# Autodesk Inventor assembly: MaleHeaderPin_1x2
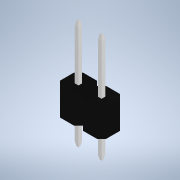
[picture p0: Inventor's stored thumbnail of the model, 180x180]
Saved by Autodesk Inventor 2021 (Build 250183000, 183)
## iProperties
Created: 2020-01-06
Part Number: MaleHeaderPin_1x2
Document SubType Name: Assembly
Designer: ermoz
Author: ermoz
## Documents named in this file (2)
- D:\Moje Wyczyny\My_Poor_Projects\Sneak100_MiniSumo\minisumo-sneak100\mechanics\PreMadeParts\MaleHeaderPin_1x2.iam
- D:\Moje Wyczyny\My_Poor_Projects\Sneak100_MiniSumo\minisumo-sneak100\mechanics\PreMadeParts\MaleHeaderPin.ipt
## Components (2 placed, 1 different names)
1. MaleHeaderPin:1 — Flush:1, Flush:8, Mate:1
2. MaleHeaderPin:2 — Flush:1, Flush:8, Mate:1
## Relationships (3: Flush 2, Mate 1)
- Flush:1: MaleHeaderPin:1 ↔ MaleHeaderPin:2
- Flush:8: MaleHeaderPin:1 ↔ MaleHeaderPin:2
- Mate:1: MaleHeaderPin:1 ↔ MaleHeaderPin:2
